# Autodesk Inventor assembly: Ford escort mk 1 & 2 steering rack
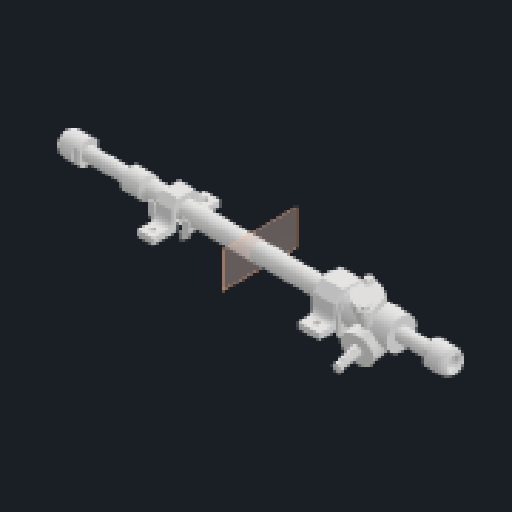
[picture p0: Inventor's stored thumbnail of the model, 512x512]
Saved by Autodesk Inventor 2025.3 (Build 293356000, 356)
## iProperties
Created: 2012-05-11
Part Number: Ford escort mk 1 & 2 steering rack
Description: STEP AP203
Document SubType Name: Assembly
Designer: VianaCC
Title: Ford escort mk 1 & 2 steering rack.STEP
Revision Number: ANY
Sending System: SolidWorks 2012
Preprocessor: SwSTEP 2.0
## Documents named in this file (5)
- C:\Users\vianacc\Documents\GitHub\utv_startup\products\utv\steering\cad\reference\Ford escort mk 1 & 2 steering rack\Ford escort mk 1 & 2 steering rack\Ford escort mk 1 & 2 steering rack.iam
- C:\Users\vianacc\Documents\GitHub\utv_startup\products\utv\steering\cad\reference\Ford escort mk 1 & 2 steering rack\Ford escort mk 1 & 2 steering rack\X7-8061-1001.ipt
- C:\Users\vianacc\Documents\GitHub\utv_startup\products\utv\steering\cad\reference\Ford escort mk 1 & 2 steering rack\Ford escort mk 1 & 2 steering rack\X7-8061-1002.ipt
- C:\Users\vianacc\Documents\GitHub\utv_startup\products\utv\steering\cad\reference\Ford escort mk 1 & 2 steering rack\Ford escort mk 1 & 2 steering rack\X7-8063-1001.ipt
- C:\Users\vianacc\Documents\GitHub\utv_startup\products\utv\steering\cad\reference\Ford escort mk 1 & 2 steering rack\Ford escort mk 1 & 2 steering rack\X7-8063-1002.ipt
## Components (4 placed, 4 different names)
1. X7-8061-1001_1
2. X7-8061-1002_2
3. X7-8063-1001_3 — Symmetry:1
4. X7-8063-1002_4 — Symmetry:1
## Relationships (1: Symmetry 1)
- Symmetry:1: X7-8063-1001_3 ↔ X7-8063-1002_4
